# Autodesk Inventor assembly: PCB Component
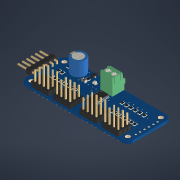
[picture p0: Inventor's stored thumbnail of the model, 180x180]
Saved by Autodesk Inventor 2021 (Build 250183000, 183)
## iProperties
Created: 2021-01-19
Part Number: PCB Component
Document SubType Name: Assembly
Designer: User
Author: User
## Documents named in this file (11)
- D:\SynologyDrive\tcodev\tco-cad\common\adafruit_pca9685\adafruit_pca9685.iam
- D:\SynologyDrive\tcodev\tco-cad\common\adafruit_pca9685\Board.ipt
- D:\SynologyDrive\tcodev\tco-cad\common\kicad_packages_3d\TSSOP-28_4.4x9.7mm_P0.65mm.ipt
- D:\SynologyDrive\tcodev\tco-cad\common\kicad_packages_3d\R_0805_2012Metric.ipt
- D:\SynologyDrive\tcodev\tco-cad\common\kicad_packages_3d\C_0805_2012Metric.ipt
- D:\SynologyDrive\tcodev\tco-cad\common\kicad_packages_3d\TerminalBlock_Phoenix_PT-1,5-2-3.5-H_1x02_P3.50mm_Horizontal.ipt
- D:\SynologyDrive\tcodev\tco-cad\common\kicad_packages_3d\SOT-23.ipt
- D:\SynologyDrive\tcodev\tco-cad\common\kicad_packages_3d\LED_0805_2012Metric.ipt
- D:\SynologyDrive\tcodev\tco-cad\common\kicad_packages_3d\CP_Radial_D8.0mm_P3.50mm.ipt
- D:\SynologyDrive\tcodev\tco-cad\common\kicad_packages_3d\PinHeader_1x06_P2.54mm_Horizontal.ipt
- D:\SynologyDrive\tcodev\tco-cad\common\kicad_packages_3d\PinHeader_1x04_P2.54mm_Vertical.ipt
## Components (46 placed, 10 different names)
1. Board:1 — Mate:1, Mate:2, Mate:3, Mate:4, Angle:1, Mate:5, Rigid:9, Rigid:10, Rigid:11, Rigid:12, Rigid:13
2. TSSOP-28_4.4x9.7mm_P0.65mm:1
3. R_0805_2012Metric:1
4. R_0805_2012Metric:2
5. R_0805_2012Metric:3
6. R_0805_2012Metric:4
7. R_0805_2012Metric:5
8. R_0805_2012Metric:6
9. C_0805_2012Metric:1
10. R_0805_2012Metric:7
11. R_0805_2012Metric:8
12. R_0805_2012Metric:9
13. R_0805_2012Metric:10
14. R_0805_2012Metric:11
15. R_0805_2012Metric:12
16. R_0805_2012Metric:13
17. R_0805_2012Metric:14
18. R_0805_2012Metric:15
19. R_0805_2012Metric:16
20. R_0805_2012Metric:17
21. R_0805_2012Metric:18
22. R_0805_2012Metric:19
23. R_0805_2012Metric:20
24. R_0805_2012Metric:22
25. R_0805_2012Metric:21
26. R_0805_2012Metric:23
27. R_0805_2012Metric:24
28. R_0805_2012Metric:25
29. R_0805_2012Metric:26
30. TerminalBlock_Phoenix_PT-1,5-2-3.5-H_1x02_P3.50mm_Horizontal:1 — Mate:1, Mate:2, Mate:3
31. SOT-23:1
32. LED_0805_2012Metric:1
33. CP_Radial_D8.0mm_P3.50mm:1 — Mate:4, Angle:1, Mate:5
34. PinHeader_1x06_P2.54mm_Horizontal:1 — Rigid:13
35. PinHeader_1x04_P2.54mm_Vertical:1 — Rigid:1, Rigid:9
36. PinHeader_1x04_P2.54mm_Vertical:2 — Rigid:1, Rigid:2
37. PinHeader_1x04_P2.54mm_Vertical:3 — Rigid:2
38. PinHeader_1x04_P2.54mm_Vertical:4 — Rigid:3, Rigid:10
39. PinHeader_1x04_P2.54mm_Vertical:5 — Rigid:3, Rigid:4
40. PinHeader_1x04_P2.54mm_Vertical:6 — Rigid:4
41. PinHeader_1x04_P2.54mm_Vertical:7 — Rigid:5, Rigid:11
42. PinHeader_1x04_P2.54mm_Vertical:8 — Rigid:5, Rigid:6
43. PinHeader_1x04_P2.54mm_Vertical:9 — Rigid:6
44. PinHeader_1x04_P2.54mm_Vertical:10 — Rigid:7, Rigid:12
45. PinHeader_1x04_P2.54mm_Vertical:11 — Rigid:7, Rigid:8
46. PinHeader_1x04_P2.54mm_Vertical:12 — Rigid:8
## Relationships (19: WeldJoint 13, Mate 5, Angle 1)
- Mate:1: Board:1 ↔ TerminalBlock_Phoenix_PT-1,5-2-3.5-H_1x02_P3.50mm_Horizontal:1
- Mate:2: Board:1 ↔ TerminalBlock_Phoenix_PT-1,5-2-3.5-H_1x02_P3.50mm_Horizontal:1
- Mate:3: Board:1 ↔ TerminalBlock_Phoenix_PT-1,5-2-3.5-H_1x02_P3.50mm_Horizontal:1
- Mate:4: Board:1 ↔ CP_Radial_D8.0mm_P3.50mm:1
- Angle:1 (0 deg): Board:1 ↔ CP_Radial_D8.0mm_P3.50mm:1
- Mate:5: Board:1 ↔ CP_Radial_D8.0mm_P3.50mm:1
- Rigid:1 [WeldJoint]: PinHeader_1x04_P2.54mm_Vertical:1 ↔ PinHeader_1x04_P2.54mm_Vertical:2
- Rigid:2 [WeldJoint]: PinHeader_1x04_P2.54mm_Vertical:2 ↔ PinHeader_1x04_P2.54mm_Vertical:3
- Rigid:3 [WeldJoint]: PinHeader_1x04_P2.54mm_Vertical:4 ↔ PinHeader_1x04_P2.54mm_Vertical:5
- Rigid:4 [WeldJoint]: PinHeader_1x04_P2.54mm_Vertical:5 ↔ PinHeader_1x04_P2.54mm_Vertical:6
- Rigid:5 [WeldJoint]: PinHeader_1x04_P2.54mm_Vertical:7 ↔ PinHeader_1x04_P2.54mm_Vertical:8
- Rigid:6 [WeldJoint]: PinHeader_1x04_P2.54mm_Vertical:8 ↔ PinHeader_1x04_P2.54mm_Vertical:9
- Rigid:7 [WeldJoint]: PinHeader_1x04_P2.54mm_Vertical:10 ↔ PinHeader_1x04_P2.54mm_Vertical:11
- Rigid:8 [WeldJoint]: PinHeader_1x04_P2.54mm_Vertical:11 ↔ PinHeader_1x04_P2.54mm_Vertical:12
- Rigid:9 [WeldJoint] (-3 mm): Board:1 ↔ PinHeader_1x04_P2.54mm_Vertical:1
- Rigid:10 [WeldJoint] (-3 mm): Board:1 ↔ PinHeader_1x04_P2.54mm_Vertical:4
- Rigid:11 [WeldJoint] (-3 mm): Board:1 ↔ PinHeader_1x04_P2.54mm_Vertical:7
- Rigid:12 [WeldJoint] (-3 mm): Board:1 ↔ PinHeader_1x04_P2.54mm_Vertical:10
- Rigid:13 [WeldJoint] (-3 mm): Board:1 ↔ PinHeader_1x06_P2.54mm_Horizontal:1
